# Autodesk Inventor assembly: Drive Pod
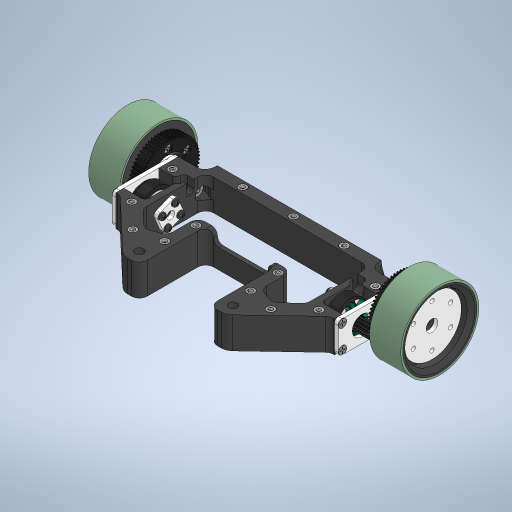
[picture p0: Inventor's stored thumbnail of the model, 512x512]
Saved by Autodesk Inventor 2023.2 (Build 272271000, 271)
## iProperties
Created: 2023-06-26
Part Number: Drive Pod
Document SubType Name: Assembly
Designer: Nathan Cai
Mass: 396.365 g
Surface Area: 1784.74 cm^2
Volume: 302.184 cm^3
Density: 1.31167 g/cm^3
Author: Nathan Cai
## Documents named in this file (32)
- E:\Documents\Inventor\Law - V1.0\Pinion Pod V1\Drive Pod.iam
- E:\Documents\Inventor\Law - V1.0\Pinion Pod V1\Just 'Cuz 2306.5 1000kV Motor v6\Just 'Cuz 2306.5 1000kV Motor v6_TOP.iam
- E:\Documents\Inventor\Law - V1.0\Pinion Pod V1\Just+Cuz+Pinion+Gear+(M0\Just+Cuz+Pinion+Gear+(M0.iam
- E:\Documents\Inventor\Law - V1.0\Pinion Pod V1\Temp - Pinion.ipt
- E:\Documents\Inventor\Law - V1.0\Pinion Pod V1\Temp - Gear.ipt
- E:\Documents\Inventor\Law - V1.0\Pinion Pod V1\Temp - Wheel.ipt
- E:\Documents\Inventor\Law - V1.0\Pinion Pod V1\Drive Pod\Design Accelerator\Spur Gears1.iam
- E:\Documents\Inventor\Law - V1.0\Pinion Pod V1\91259A542_Alloy Steel Shoulder Screw\91259A542_Alloy Steel Shoulder Screw.ipt
- E:\Documents\Inventor\Law - V1.0\Pinion Pod V1\Pod.ipt
- E:\Documents\Inventor\Law - V1.0\Pinion Pod V1\90631A011_Low-Strength Steel Nylon-Insert Locknut\90631A011_Low-Strength Steel Nylon-Insert Locknut.ipt
- E:\Documents\Inventor\Law - V1.0\Pinion Pod V1\Temp - Tire.ipt
- E:\Documents\Inventor\Law - V1.0\Pinion Pod V1\Standoff 1in.ipt
- E:\Documents\Inventor\Law - V1.0\Pinion Pod V1\Brace.ipt
- E:\Documents\Inventor\Content Center Files\R2023\en-US\ISO 7045  H\ISO 7045 - M3 x 8_ - 4.8 - H - ISO.ipt
- E:\Documents\Inventor\Law - V1.0\Face PLate.ipt
- E:\Documents\Inventor\Content Center Files\R2023\en-US\ANSI B18.6.3(12)\ANSI B18.6.3 - 6-32 UNC - 0.3125(15_).ipt
- E:\Documents\Inventor\Law - V1.0\Standoff 1in.ipt
- E:\Documents\Inventor\Law - V1.0\Pinion Pod V1\MIR\Just 'Cuz 2306.5 1000kV Motor v6_TOP_MIR.iam
- E:\Documents\Inventor\Law - V1.0\Pinion Pod V1\MIR\Just+Cuz+Pinion+Gear+(M0_MIR.iam
- E:\Documents\Inventor\Law - V1.0\Pinion Pod V1\MIR\Temp - Wheel_MIR.ipt
- E:\Documents\Inventor\Law - V1.0\Pinion Pod V1\MIR\Temp - Tire_MIR.ipt
- E:\Documents\Inventor\Law - V1.0\Pinion Pod V1\MIR\Spur Gears1_MIR.iam
- E:\Documents\Inventor\Law - V1.0\Pinion Pod V1\MIR\91259A542_Alloy Steel Shoulder Screw_MIR.ipt
- E:\Documents\Inventor\Law - V1.0\Pinion Pod V1\MIR\90631A011_Low-Strength Steel Nylon-Insert Locknut_MIR.ipt
- E:\Documents\Inventor\Law - V1.0\Pinion Pod V1\MIR\Standoff 1in_MIR.ipt
- E:\Documents\Inventor\Law - V1.0\Pinion Pod V1\MIR\Brace_MIR.ipt
- E:\Documents\Inventor\Law - V1.0\Pinion Pod V1\MIR\Face PLate_MIR.ipt
- E:\Documents\Inventor\Law - V1.0\Pinion Pod V1\MIR\Standoff 1in_MIR1.ipt
- E:\Documents\Inventor\Law - V1.0\Bushing.ipt
- E:\Documents\Inventor\Content Center Files\R2023\en-US\ANSI B18.6.3(27)\ANSI B18.6.3 - 6-32 UNC - 0.75(11).ipt
- E:\Documents\Inventor\Law - V1.0\Pinion Pod V1\Wheel Cover.ipt
- E:\Documents\Inventor\Law - V1.0\Pinion Pod V1\Export\Spacer.ipt
## Components (71 placed, 30 different names)
1. Just 'Cuz 2306.5 1000kV Motor v6_TOP:1 [sub-assembly] — Mate:1, Mate:2, Mate:3, Flush:4, Mate:93, Mate:94
2. Just+Cuz+Pinion+Gear+(M0:1 [sub-assembly] — Mate:1, Mate:2, Flush:1, Flush:3
3. Temp - Pinion:1 — Tangent:1, Mate:3, Flush:1, Flush:2, Mate:38
4. Temp - Gear:1 — Tangent:1, Flush:2, Mate:5, Mate:37
5. Temp - Wheel:1 — Mate:5, Mate:16, Mate:92, Flush:18, Mate:108, Mate:133, Mate:134
6. Spur Gears:1 [sub-assembly] — Flush:3, Mate:8, Mate:16, Mate:37, Mate:38, Mate:83, Mate:88, Mate:89, Mate:108, Mate:109, Mate:110, Mate:111, Mate:112, Mate:113, Mate:114, Mate:115, Mate:116, Mate:117, Mate:118, Mate:119, Mate:120
7. 91259A542_Alloy Steel Shoulder Screw:1 — Mate:8, Mate:10, Mate:13, Mate:19, Mate:48, Mate:83
8. Pod:1 — Mate:10, Mate:15, Mate:17, Mate:18, Mate:21, Mate:22, Mate:23, Mate:24, Mate:25, Flush:6, Flush:7, Mate:47, Flush:8, Mate:54, Mate:55, Mate:56, Mate:57, Flush:9, Flush:10, Flush:11, Flush:12, Mate:58, Flush:13, Flush:17, Mate:93, Mate:94, Mate:95, Mate:96, Mate:97, Mate:98, Mate:99
9. 90631A011_Low-Strength Steel Nylon-Insert Locknut:1 — Mate:17, Mate:18, Mate:19
10. Standoff 1in:1 — Mate:21, Flush:6
11. Standoff 1in:2 — Mate:22, Flush:7
12. Brace:1 — Mate:23, Mate:24, Mate:25, Mate:100, Mate:101, Mate:102, Mate:103, Mate:104, Mate:105, Mate:106, Mate:107
13. Face PLate:1 — Mate:47, Mate:48, Flush:8, Mate:49, Mate:50, Mate:51, Mate:52, Mate:53
14. Cross Recessed Flat Countersunk Head Machine Screw - Type I - Inch 6-32 x 5/16:1 — Mate:49
15. Cross Recessed Flat Countersunk Head Machine Screw - Type I - Inch 6-32 x 5/16:2 — Mate:50
16. Cross Recessed Flat Countersunk Head Machine Screw - Type I - Inch 6-32 x 5/16:3 — Mate:51
17. Cross Recessed Flat Countersunk Head Machine Screw - Type I - Inch 6-32 x 5/16:4 — Mate:52
18. Cross Recessed Flat Countersunk Head Machine Screw - Type I - Inch 6-32 x 5/16:5 — Mate:53
19. Standoff 1in:3 — Mate:57, Flush:12
20. Standoff 1in:4 — Mate:56, Flush:11
21. Standoff 1in:5 — Mate:54, Flush:9
22. Standoff 1in:6 — Mate:55, Flush:10
23. Bushing:2 — Mate:90, Mate:91
24. Cross Recessed Truss Head Machine Screw - Type I - Inch No. 6 - 32 - 3/4:1 — Mate:109, Mate:110
25. Cross Recessed Truss Head Machine Screw - Type I - Inch No. 6 - 32 - 3/4:2 — Mate:111, Mate:112
26. Cross Recessed Truss Head Machine Screw - Type I - Inch No. 6 - 32 - 3/4:3 — Mate:113, Mate:114
27. Cross Recessed Truss Head Machine Screw - Type I - Inch No. 6 - 32 - 3/4:4 — Mate:115, Mate:116
28. Cross Recessed Truss Head Machine Screw - Type I - Inch No. 6 - 32 - 3/4:5 — Mate:117, Mate:118
29. Cross Recessed Truss Head Machine Screw - Type I - Inch No. 6 - 32 - 3/4:6 — Mate:119, Mate:120
30. Wheel Cover:1 — Mate:133, Mate:134
31. Wheel Cover:2 — Mate:135, Mate:136
32. Spacer:1
33. Bushing:1 — Mate:88, Mate:89
34. Temp - Tire:2 — Mate:92, Flush:18
35. ISO 7045 H M3 x 8 - 4.8 - H:1 — Mate:100, Mate:101
36. ISO 7045 H M3 x 8 - 4.8 - H:9 — Mate:102, Mate:103
37. ISO 7045 H M3 x 8 - 4.8 - H:10 — Mate:104, Mate:105
38. ISO 7045 H M3 x 8 - 4.8 - H:11 — Mate:106, Mate:107
39. Cross Recessed Truss Head Machine Screw - Type I - Inch No. 6 - 32 - 3/4:7 — Mate:121, Mate:122
40. Cross Recessed Truss Head Machine Screw - Type I - Inch No. 6 - 32 - 3/4:8 — Mate:123, Mate:124
41. Cross Recessed Truss Head Machine Screw - Type I - Inch No. 6 - 32 - 3/4:9 — Mate:125, Mate:126
42. Cross Recessed Truss Head Machine Screw - Type I - Inch No. 6 - 32 - 3/4:10 — Mate:127, Mate:128
43. Cross Recessed Truss Head Machine Screw - Type I - Inch No. 6 - 32 - 3/4:11 — Mate:129, Mate:130
44. Cross Recessed Truss Head Machine Screw - Type I - Inch No. 6 - 32 - 3/4:12 — Mate:131, Mate:132
45. Standoff 1in:7 — Mate:58, Flush:13
46. Just 'Cuz 2306.5 1000kV Motor v6_TOP_MIR:1 [sub-assembly] — Flush:14, Mate:60, Mate:61, Mate:98, Mate:99
47. Just+Cuz+Pinion+Gear+(M0_MIR:1 [sub-assembly] — Mate:60, Mate:61, Flush:15
48. Temp - Pinion:2
49. Temp - Gear:2
50. Temp - Wheel_MIR:1 — Mate:62, Flush:16, Mate:68, Mate:85, Mate:86, Mate:87, Mate:135, Mate:136
51. Temp - Tire_MIR:1 — Flush:16, Mate:68
52. Spur Gears1_MIR:1 [sub-assembly] — Mate:62, Flush:15, Mate:65, Mate:66, Mate:85, Mate:86, Mate:90, Mate:91, Mate:121, Mate:122, Mate:123, Mate:124, Mate:125, Mate:126, Mate:127, Mate:128, Mate:129, Mate:130, Mate:131, Mate:132
53. 91259A542_Alloy Steel Shoulder Screw_MIR:1 — Mate:64, Mate:65, Mate:66, Mate:67, Mate:77, Mate:87
54. 90631A011_Low-Strength Steel Nylon-Insert Locknut_MIR:1 — Mate:67
55. Standoff 1in_MIR:1
56. Standoff 1in_MIR:2
57. Brace_MIR:1 — Mate:69, Mate:70, Mate:71, Mate:72, Mate:73, Mate:74, Mate:75, Mate:76, Mate:95, Mate:97
58. ISO 7045 H M3 x 8 - 4.8 - H:5 — Mate:69, Mate:70, Mate:96
59. ISO 7045 H M3 x 8 - 4.8 - H:6 — Mate:71, Mate:72
60. ISO 7045 H M3 x 8 - 4.8 - H:7 — Mate:73, Mate:74
61. ISO 7045 H M3 x 8 - 4.8 - H:8 — Mate:75, Mate:76
62. Face PLate_MIR:1 — Mate:77, Mate:78, Mate:79, Mate:80, Mate:81, Mate:82, Flush:17
63. Cross Recessed Flat Countersunk Head Machine Screw - Type I - Inch 6-32 x 5/16:6 — Mate:78
64. Cross Recessed Flat Countersunk Head Machine Screw - Type I - Inch 6-32 x 5/16:7 — Mate:79
65. Cross Recessed Flat Countersunk Head Machine Screw - Type I - Inch 6-32 x 5/16:8 — Mate:80
66. Cross Recessed Flat Countersunk Head Machine Screw - Type I - Inch 6-32 x 5/16:9 — Mate:81
67. Cross Recessed Flat Countersunk Head Machine Screw - Type I - Inch 6-32 x 5/16:10 — Mate:82
68. Standoff 1in_MIR1:1
69. Standoff 1in_MIR1:2
70. Standoff 1in_MIR1:3
71. Standoff 1in_MIR1:4
## Relationships (124: Mate 106, Flush 17, Tangent 1)
- Mate:1: Just 'Cuz 2306.5 1000kV Motor v6_TOP:1 ↔ Just+Cuz+Pinion+Gear+(M0:1
- Mate:2: Just 'Cuz 2306.5 1000kV Motor v6_TOP:1 ↔ Just+Cuz+Pinion+Gear+(M0:1
- Tangent:1: Temp - Pinion:1 ↔ Temp - Gear:1
- Mate:3: Just 'Cuz 2306.5 1000kV Motor v6_TOP:1 ↔ Temp - Pinion:1
- Flush:1: Just+Cuz+Pinion+Gear+(M0:1 ↔ Temp - Pinion:1
- Flush:2: Temp - Pinion:1 ↔ Temp - Gear:1
- Mate:5: Temp - Gear:1 ↔ Temp - Wheel:1
- Flush:3 (-1 mm): Just+Cuz+Pinion+Gear+(M0:1 ↔ Spur Gears:1
- Mate:8: Spur Gears:1 ↔ 91259A542_Alloy Steel Shoulder Screw:1
- Mate:10: 91259A542_Alloy Steel Shoulder Screw:1 ↔ Pod:1
- Flush:4: Just 'Cuz 2306.5 1000kV Motor v6_TOP:1
- Mate:13: 91259A542_Alloy Steel Shoulder Screw:1
- Mate:15: Pod:1
- Mate:16: Temp - Wheel:1 ↔ Spur Gears:1
- Mate:17: Pod:1 ↔ 90631A011_Low-Strength Steel Nylon-Insert Locknut:1
- Mate:18: Pod:1 ↔ 90631A011_Low-Strength Steel Nylon-Insert Locknut:1
- Mate:19: 91259A542_Alloy Steel Shoulder Screw:1 ↔ 90631A011_Low-Strength Steel Nylon-Insert Locknut:1
- Mate:21: Pod:1 ↔ Standoff 1in:1
- Mate:22: Pod:1 ↔ Standoff 1in:2
- Mate:23: Pod:1 ↔ Brace:1
- Mate:24: Pod:1 ↔ Brace:1
- Mate:25: Pod:1 ↔ Brace:1
- Mate:37: Temp - Gear:1 ↔ Spur Gears:1
- Mate:38: Temp - Pinion:1 ↔ Spur Gears:1
- Flush:6: Pod:1 ↔ Standoff 1in:1
- Flush:7: Pod:1 ↔ Standoff 1in:2
- Mate:47: Pod:1 ↔ Face PLate:1
- Mate:48: 91259A542_Alloy Steel Shoulder Screw:1 ↔ Face PLate:1
- Flush:8: Pod:1 ↔ Face PLate:1
- Mate:49: Face PLate:1 ↔ Cross Recessed Flat Countersunk Head Machine Screw - Type I - Inch 6-32 x 5/16:1
- Mate:50: Face PLate:1 ↔ Cross Recessed Flat Countersunk Head Machine Screw - Type I - Inch 6-32 x 5/16:2
- Mate:51: Face PLate:1 ↔ Cross Recessed Flat Countersunk Head Machine Screw - Type I - Inch 6-32 x 5/16:3
- Mate:52: Face PLate:1 ↔ Cross Recessed Flat Countersunk Head Machine Screw - Type I - Inch 6-32 x 5/16:4
- Mate:53: Face PLate:1 ↔ Cross Recessed Flat Countersunk Head Machine Screw - Type I - Inch 6-32 x 5/16:5
- Mate:54: Pod:1 ↔ Standoff 1in:5
- Mate:55: Pod:1 ↔ Standoff 1in:6
- Mate:56: Pod:1 ↔ Standoff 1in:4
- Mate:57: Pod:1 ↔ Standoff 1in:3
- Flush:9: Pod:1 ↔ Standoff 1in:5
- Flush:10: Pod:1 ↔ Standoff 1in:6
- Flush:11: Pod:1 ↔ Standoff 1in:4
- Flush:12: Pod:1 ↔ Standoff 1in:3
- Mate:58: Pod:1 ↔ Standoff 1in:7
- Flush:13: Pod:1 ↔ Standoff 1in:7
- Flush:14: Just 'Cuz 2306.5 1000kV Motor v6_TOP_MIR:1
- Mate:60: Just 'Cuz 2306.5 1000kV Motor v6_TOP_MIR:1 ↔ Just+Cuz+Pinion+Gear+(M0_MIR:1
- Mate:61: Just 'Cuz 2306.5 1000kV Motor v6_TOP_MIR:1 ↔ Just+Cuz+Pinion+Gear+(M0_MIR:1
- Mate:62: Temp - Wheel_MIR:1 ↔ Spur Gears1_MIR:1
- Flush:15 (-1 mm): Just+Cuz+Pinion+Gear+(M0_MIR:1 ↔ Spur Gears1_MIR:1
- Mate:64: 91259A542_Alloy Steel Shoulder Screw_MIR:1
- Mate:65 (3.175 mm): Spur Gears1_MIR:1 ↔ 91259A542_Alloy Steel Shoulder Screw_MIR:1
- Mate:66: Spur Gears1_MIR:1 ↔ 91259A542_Alloy Steel Shoulder Screw_MIR:1
- Mate:67: 91259A542_Alloy Steel Shoulder Screw_MIR:1 ↔ 90631A011_Low-Strength Steel Nylon-Insert Locknut_MIR:1
- Flush:16: Temp - Wheel_MIR:1 ↔ Temp - Tire_MIR:1
- Mate:68: Temp - Wheel_MIR:1 ↔ Temp - Tire_MIR:1
- Mate:69: Brace_MIR:1 ↔ ISO 7045 H M3 x 8 - 4.8 - H:5
- Mate:70: Brace_MIR:1 ↔ ISO 7045 H M3 x 8 - 4.8 - H:5
- Mate:71: Brace_MIR:1 ↔ ISO 7045 H M3 x 8 - 4.8 - H:6
- Mate:72: Brace_MIR:1 ↔ ISO 7045 H M3 x 8 - 4.8 - H:6
- Mate:73: Brace_MIR:1 ↔ ISO 7045 H M3 x 8 - 4.8 - H:7
- Mate:74: Brace_MIR:1 ↔ ISO 7045 H M3 x 8 - 4.8 - H:7
- Mate:75: Brace_MIR:1 ↔ ISO 7045 H M3 x 8 - 4.8 - H:8
- Mate:76: Brace_MIR:1 ↔ ISO 7045 H M3 x 8 - 4.8 - H:8
- Mate:77: 91259A542_Alloy Steel Shoulder Screw_MIR:1 ↔ Face PLate_MIR:1
- Mate:78: Face PLate_MIR:1 ↔ Cross Recessed Flat Countersunk Head Machine Screw - Type I - Inch 6-32 x 5/16:6
- Mate:79: Face PLate_MIR:1 ↔ Cross Recessed Flat Countersunk Head Machine Screw - Type I - Inch 6-32 x 5/16:7
- Mate:80: Face PLate_MIR:1 ↔ Cross Recessed Flat Countersunk Head Machine Screw - Type I - Inch 6-32 x 5/16:8
- Mate:81: Face PLate_MIR:1 ↔ Cross Recessed Flat Countersunk Head Machine Screw - Type I - Inch 6-32 x 5/16:9
- Mate:82: Face PLate_MIR:1 ↔ Cross Recessed Flat Countersunk Head Machine Screw - Type I - Inch 6-32 x 5/16:10
- Mate:83 (3.175 mm): Spur Gears:1 ↔ 91259A542_Alloy Steel Shoulder Screw:1
- Mate:85: Temp - Wheel_MIR:1 ↔ Spur Gears1_MIR:1
- Mate:86: Temp - Wheel_MIR:1 ↔ Spur Gears1_MIR:1
- Mate:87: Temp - Wheel_MIR:1 ↔ 91259A542_Alloy Steel Shoulder Screw_MIR:1
- Flush:17: Pod:1 ↔ Face PLate_MIR:1
- Mate:88: Spur Gears:1 ↔ Bushing:1
- Mate:89: Spur Gears:1 ↔ Bushing:1
- Mate:90: Bushing:2 ↔ Spur Gears1_MIR:1
- Mate:91: Bushing:2 ↔ Spur Gears1_MIR:1
- Mate:92: Temp - Wheel:1 ↔ Temp - Tire:2
- Flush:18: Temp - Wheel:1 ↔ Temp - Tire:2
- Mate:93: Just 'Cuz 2306.5 1000kV Motor v6_TOP:1 ↔ Pod:1
- Mate:94: Just 'Cuz 2306.5 1000kV Motor v6_TOP:1 ↔ Pod:1
- Mate:95: Pod:1 ↔ Brace_MIR:1
- Mate:96: Pod:1 ↔ ISO 7045 H M3 x 8 - 4.8 - H:5
- Mate:97: Pod:1 ↔ Brace_MIR:1
- Mate:98: Pod:1 ↔ Just 'Cuz 2306.5 1000kV Motor v6_TOP_MIR:1
- Mate:99: Pod:1 ↔ Just 'Cuz 2306.5 1000kV Motor v6_TOP_MIR:1
- Mate:100: Brace:1 ↔ ISO 7045 H M3 x 8 - 4.8 - H:1
- Mate:101: Brace:1 ↔ ISO 7045 H M3 x 8 - 4.8 - H:1
- Mate:102: Brace:1 ↔ ISO 7045 H M3 x 8 - 4.8 - H:9
- Mate:103: Brace:1 ↔ ISO 7045 H M3 x 8 - 4.8 - H:9
- Mate:104: Brace:1 ↔ ISO 7045 H M3 x 8 - 4.8 - H:10
- Mate:105: Brace:1 ↔ ISO 7045 H M3 x 8 - 4.8 - H:10
- Mate:106: Brace:1 ↔ ISO 7045 H M3 x 8 - 4.8 - H:11
- Mate:107: Brace:1 ↔ ISO 7045 H M3 x 8 - 4.8 - H:11
- Mate:108: Temp - Wheel:1 ↔ Spur Gears:1
- Mate:109: Spur Gears:1 ↔ Cross Recessed Truss Head Machine Screw - Type I - Inch No. 6 - 32 - 3/4:1
- Mate:110: Spur Gears:1 ↔ Cross Recessed Truss Head Machine Screw - Type I - Inch No. 6 - 32 - 3/4:1
- Mate:111: Spur Gears:1 ↔ Cross Recessed Truss Head Machine Screw - Type I - Inch No. 6 - 32 - 3/4:2
- Mate:112: Spur Gears:1 ↔ Cross Recessed Truss Head Machine Screw - Type I - Inch No. 6 - 32 - 3/4:2
- Mate:113: Spur Gears:1 ↔ Cross Recessed Truss Head Machine Screw - Type I - Inch No. 6 - 32 - 3/4:3
- Mate:114: Spur Gears:1 ↔ Cross Recessed Truss Head Machine Screw - Type I - Inch No. 6 - 32 - 3/4:3
- Mate:115: Spur Gears:1 ↔ Cross Recessed Truss Head Machine Screw - Type I - Inch No. 6 - 32 - 3/4:4
- Mate:116: Spur Gears:1 ↔ Cross Recessed Truss Head Machine Screw - Type I - Inch No. 6 - 32 - 3/4:4
- Mate:117: Spur Gears:1 ↔ Cross Recessed Truss Head Machine Screw - Type I - Inch No. 6 - 32 - 3/4:5
- Mate:118: Spur Gears:1 ↔ Cross Recessed Truss Head Machine Screw - Type I - Inch No. 6 - 32 - 3/4:5
- Mate:119: Spur Gears:1 ↔ Cross Recessed Truss Head Machine Screw - Type I - Inch No. 6 - 32 - 3/4:6
- Mate:120: Spur Gears:1 ↔ Cross Recessed Truss Head Machine Screw - Type I - Inch No. 6 - 32 - 3/4:6
- Mate:121: Cross Recessed Truss Head Machine Screw - Type I - Inch No. 6 - 32 - 3/4:7 ↔ Spur Gears1_MIR:1
- Mate:122: Cross Recessed Truss Head Machine Screw - Type I - Inch No. 6 - 32 - 3/4:7 ↔ Spur Gears1_MIR:1
- Mate:123: Cross Recessed Truss Head Machine Screw - Type I - Inch No. 6 - 32 - 3/4:8 ↔ Spur Gears1_MIR:1
- Mate:124: Cross Recessed Truss Head Machine Screw - Type I - Inch No. 6 - 32 - 3/4:8 ↔ Spur Gears1_MIR:1
- Mate:125: Cross Recessed Truss Head Machine Screw - Type I - Inch No. 6 - 32 - 3/4:9 ↔ Spur Gears1_MIR:1
- Mate:126: Cross Recessed Truss Head Machine Screw - Type I - Inch No. 6 - 32 - 3/4:9 ↔ Spur Gears1_MIR:1
- Mate:127: Cross Recessed Truss Head Machine Screw - Type I - Inch No. 6 - 32 - 3/4:10 ↔ Spur Gears1_MIR:1
- Mate:128: Cross Recessed Truss Head Machine Screw - Type I - Inch No. 6 - 32 - 3/4:10 ↔ Spur Gears1_MIR:1
- Mate:129: Cross Recessed Truss Head Machine Screw - Type I - Inch No. 6 - 32 - 3/4:11 ↔ Spur Gears1_MIR:1
- Mate:130: Cross Recessed Truss Head Machine Screw - Type I - Inch No. 6 - 32 - 3/4:11 ↔ Spur Gears1_MIR:1
- Mate:131: Cross Recessed Truss Head Machine Screw - Type I - Inch No. 6 - 32 - 3/4:12 ↔ Spur Gears1_MIR:1
- Mate:132: Cross Recessed Truss Head Machine Screw - Type I - Inch No. 6 - 32 - 3/4:12 ↔ Spur Gears1_MIR:1
- Mate:133: Temp - Wheel:1 ↔ Wheel Cover:1
- Mate:134: Temp - Wheel:1 ↔ Wheel Cover:1
- Mate:135: Wheel Cover:2 ↔ Temp - Wheel_MIR:1
- Mate:136: Wheel Cover:2 ↔ Temp - Wheel_MIR:1
